# Autodesk Inventor assembly: StepperSystem
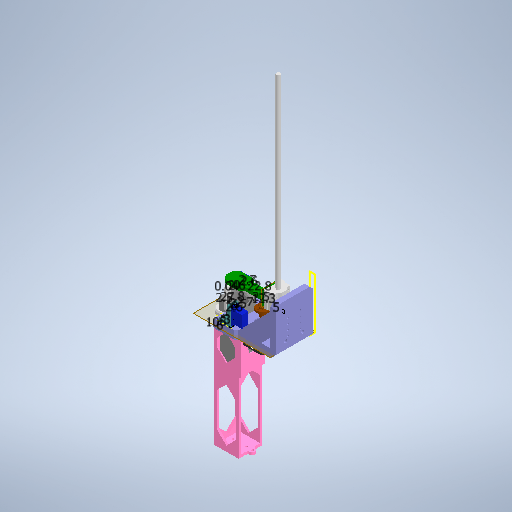
[picture p0: Inventor's stored thumbnail of the model, 512x512]
Saved by Autodesk Inventor 2025.1 (Build 291241000, 241)
## iProperties
Created: 2025-01-26
Part Number: StepperSystem
Document SubType Name: Assembly
Designer: 13156
Author: 13156
## Documents named in this file (19)
- C:\Users\13156\OneDrive - Binghamton University\Documents\GitHub\Perovskite-Automated-Synthesis-System\CAD\Pipette\StepperSystem.iam
- C:\Users\13156\OneDrive - Binghamton University\Documents\GitHub\Perovskite-Automated-Synthesis-System\CAD\Pipette\HolderWStepper.ipt
- C:\Users\13156\OneDrive - Binghamton University\Documents\GitHub\Perovskite-Automated-Synthesis-System\CAD\Non 3D Printed Parts\Linear Rails\8mm Linear Rod.ipt
- C:\Users\13156\OneDrive - Binghamton University\Documents\GitHub\Perovskite-Automated-Synthesis-System\CAD\Non 3D Printed Parts\Linear Rails\Linear Bearing 8mm Square.ipt
- C:\Users\13156\OneDrive - Binghamton University\Documents\GitHub\Perovskite-Automated-Synthesis-System\CAD\Pipette\Actuator.ipt
- C:\Users\13156\OneDrive - Binghamton University\Documents\GitHub\Perovskite-Automated-Synthesis-System\CAD\Pipette\PipetteStand.ipt
- C:\Users\13156\OneDrive - Binghamton University\Documents\GitHub\Perovskite-Automated-Synthesis-System\CAD\Non 3D Printed Parts\Motors and Servos\SG90 Servo.ipt
- C:\Users\13156\OneDrive - Binghamton University\Documents\GitHub\Perovskite-Automated-Synthesis-System\CAD\Pipette\SLEEVE.ipt
- C:\Users\13156\OneDrive - Binghamton University\Documents\GitHub\Perovskite-Automated-Synthesis-System\CAD\Non 3D Printed Parts\Leadscrew.ipt
- C:\Users\13156\OneDrive - Binghamton University\Documents\GitHub\Perovskite-Automated-Synthesis-System\CAD\Non 3D Printed Parts\Linear Rails\Linear Rod Holder SK8.ipt
- C:\Users\13156\OneDrive - Binghamton University\Documents\GitHub\Perovskite-Automated-Synthesis-System\CAD\Non 3D Printed Parts\Motors and Servos\NEMA17 Stepper Motor - 26 mm.ipt
- C:\Users\13156\OneDrive - Binghamton University\Documents\GitHub\Perovskite-Automated-Synthesis-System\CAD\Pipette\ServoHolder.ipt
- C:\Users\13156\OneDrive - Binghamton University\Documents\GitHub\Perovskite-Automated-Synthesis-System\CAD\Non 3D Printed Parts\Screws\M3x12.ipt
- C:\Users\13156\OneDrive - Binghamton University\Documents\GitHub\Perovskite-Automated-Synthesis-System\CAD\Non 3D Printed Parts\Screws\M2x8.ipt
- C:\Users\13156\OneDrive - Binghamton University\Documents\GitHub\Perovskite-Automated-Synthesis-System\CAD\Non 3D Printed Parts\Screws\M3x8.ipt
- C:\Users\13156\OneDrive - Binghamton University\Documents\GitHub\Perovskite-Automated-Synthesis-System\CAD\Pipette\HalfServoArm.ipt
- C:\Users\13156\OneDrive - Binghamton University\Documents\GitHub\Perovskite-Automated-Synthesis-System\CAD\Pipette\GrabberArmV2.ipt
- C:\Users\13156\OneDrive - Binghamton University\Documents\GitHub\Perovskite-Automated-Synthesis-System\CAD\Pipette\GrabberServoHolder.ipt
- C:\Users\13156\OneDrive - Binghamton University\Documents\GitHub\Perovskite-Automated-Synthesis-System\CAD\Pipette\EjectorArm.ipt
## Components (21 placed, 18 different names)
1. HolderWStepper:1 — Mate:9, Mate:13, Mate:14, Mate:15, Mate:16, Mate:25, Mate:26, Flush:4, Mate:46, Mate:47, Mate:50, Mate:51, Mate:54, Mate:95, Mate:100, Mate:101, Mate:102
2. 8mm Linear Rod:1 — Mate:21, Flush:4, Mate:48
3. Linear Bearing 8mm Square:1 — Mate:21, Mate:28, Mate:29, Mate:30, Mate:49
4. Actuator:1 — Mate:28, Mate:29, Mate:30, Mate:31, Mate:32, Mate:33, Mate:49
5. PipetteStand:1 — Mate:1, Mate:2, Mate:3, Mate:4, Mate:6
6. SG90 Servo:1 — Mate:98, Mate:99
7. Leadscrew:1 — Mate:31, Mate:32, Mate:33
8. Linear Rod Holder SK8:1 — Mate:13, Mate:14, Mate:15, Mate:16, Mate:48
9. SG90 Servo:3 — Mate:104, Mate:105, Mate:106, Mate:107
10. NEMA17 Stepper Motor - 26 mm:2 — Mate:9, Mate:25, Mate:26
11. SLEEVE:1 — Mate:4, Mate:6, Mate:46, Mate:47, Mate:54, Mate:90, Mate:91, Mate:92, Mate:95, Mate:103
12. ServoHolder:1 — Mate:50, Mate:51, Mate:63, Mate:64, Mate:65, Mate:66, Mate:69, Mate:70, Mate:104, Mate:105
13. M3x12:1 — Mate:63, Mate:64, Mate:70
14. M3x12:2 — Mate:65, Mate:66, Mate:69
15. M2x8:1
16. M3x8:1
17. HalfServoArm:1 — Mate:93, Mate:94, Mate:98, Mate:99
18. GrabberArmV2:1 — Mate:90, Mate:91, Mate:92, Mate:93, Mate:94, Mate:103
19. GrabberServoHolder:1 — Mate:100, Mate:101, Mate:102
20. EjectorArm:2 — Mate:108, Mate:109
21. HalfServoArm:2 — Mate:106, Mate:107, Mate:108, Mate:109
## Relationships (51: Mate 50, Flush 1)
- Mate:1: PipetteStand:1
- Mate:2: PipetteStand:1
- Mate:3: PipetteStand:1
- Mate:4: PipetteStand:1 ↔ SLEEVE:1
- Mate:6 (0.5 mm): PipetteStand:1 ↔ SLEEVE:1
- Mate:9: HolderWStepper:1 ↔ NEMA17 Stepper Motor - 26 mm:2
- Mate:13: HolderWStepper:1 ↔ Linear Rod Holder SK8:1
- Mate:14: HolderWStepper:1 ↔ Linear Rod Holder SK8:1
- Mate:15: HolderWStepper:1 ↔ Linear Rod Holder SK8:1
- Mate:16: HolderWStepper:1 ↔ Linear Rod Holder SK8:1
- Mate:21: 8mm Linear Rod:1 ↔ Linear Bearing 8mm Square:1
- Mate:25: HolderWStepper:1 ↔ NEMA17 Stepper Motor - 26 mm:2
- Mate:26: HolderWStepper:1 ↔ NEMA17 Stepper Motor - 26 mm:2
- Mate:28: Linear Bearing 8mm Square:1 ↔ Actuator:1
- Mate:29: Linear Bearing 8mm Square:1 ↔ Actuator:1
- Mate:30: Linear Bearing 8mm Square:1 ↔ Actuator:1
- Mate:31: Actuator:1 ↔ Leadscrew:1
- Mate:32: Actuator:1 ↔ Leadscrew:1
- Mate:33: Actuator:1 ↔ Leadscrew:1
- Flush:4: HolderWStepper:1 ↔ 8mm Linear Rod:1
- Mate:46: HolderWStepper:1 ↔ SLEEVE:1
- Mate:47: HolderWStepper:1 ↔ SLEEVE:1
- Mate:48: 8mm Linear Rod:1 ↔ Linear Rod Holder SK8:1
- Mate:49: Linear Bearing 8mm Square:1 ↔ Actuator:1
- Mate:50: HolderWStepper:1 ↔ ServoHolder:1
- Mate:51: HolderWStepper:1 ↔ ServoHolder:1
- Mate:54: HolderWStepper:1 ↔ SLEEVE:1
- Mate:63: ServoHolder:1 ↔ M3x12:1
- Mate:64: ServoHolder:1 ↔ M3x12:1
- Mate:65: ServoHolder:1 ↔ M3x12:2
- Mate:66: ServoHolder:1 ↔ M3x12:2
- Mate:69: ServoHolder:1 ↔ M3x12:2
- Mate:70: ServoHolder:1 ↔ M3x12:1
- Mate:90: SLEEVE:1 ↔ GrabberArmV2:1
- Mate:91: SLEEVE:1 ↔ GrabberArmV2:1
- Mate:92: SLEEVE:1 ↔ GrabberArmV2:1
- Mate:93: HalfServoArm:1 ↔ GrabberArmV2:1
- Mate:94: HalfServoArm:1 ↔ GrabberArmV2:1
- Mate:95: HolderWStepper:1 ↔ SLEEVE:1
- Mate:98: SG90 Servo:1 ↔ HalfServoArm:1
- Mate:99: SG90 Servo:1 ↔ HalfServoArm:1
- Mate:100: HolderWStepper:1 ↔ GrabberServoHolder:1
- Mate:101: HolderWStepper:1 ↔ GrabberServoHolder:1
- Mate:102: HolderWStepper:1 ↔ GrabberServoHolder:1
- Mate:103: SLEEVE:1 ↔ GrabberArmV2:1
- Mate:104: SG90 Servo:3 ↔ ServoHolder:1
- Mate:105: SG90 Servo:3 ↔ ServoHolder:1
- Mate:106: SG90 Servo:3 ↔ HalfServoArm:2
- Mate:107: SG90 Servo:3 ↔ HalfServoArm:2
- Mate:108: EjectorArm:2 ↔ HalfServoArm:2
- Mate:109: EjectorArm:2 ↔ HalfServoArm:2
